# Autodesk Inventor assembly: Assembly8
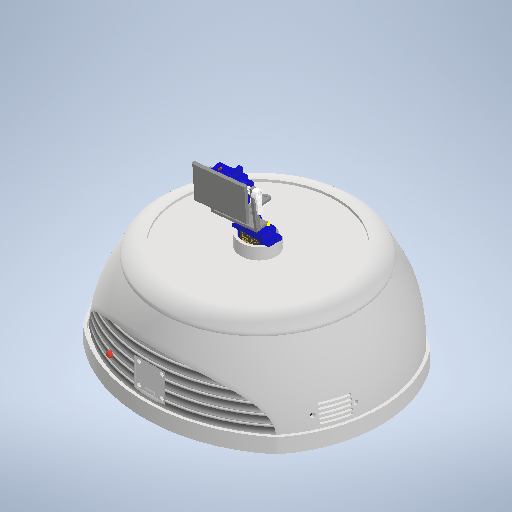
[picture p0: Inventor's stored thumbnail of the model, 512x512]
Saved by Autodesk Inventor 2025.3 (Build 293356030, 356C)
## iProperties
Created: 2026-07-17
Part Number: Assembly8
Document SubType Name: Assembly
Designer: Samuel Correa Vega
Author: Samuel Correa Vega
## Documents named in this file (12)
- C:\Users\Samuel Correa Vega\Documents\Mini-Nathan\Full Robot.iam
- C:\Users\Samuel Correa Vega\Documents\Mini-Nathan\Upper Base.ipt
- C:\Users\Samuel Correa Vega\Documents\ROBOT\Beeper buzzer 3-24V 23dia 11h leaded\Beeper buzzer 3-24V 23dia 11h leaded\Beeper buzzer 3-24V 23dia 11h leaded.ipt
- C:\Users\Samuel Correa Vega\Documents\ROBOT\SG90 - Micro Servo 9g - Tower Pro.1\SG90 - Micro Servo 9g - Tower Pro.1\SG90 - Micro Servo 9g - Tower Pro.1.ipt
- C:\Users\Samuel Correa Vega\Documents\ROBOT\SG90 - Micro Servo 9g - Tower Pro.3\SG90 - Micro Servo 9g - Tower Pro.3\SG90 - Micro Servo 9g - Tower Pro.3.ipt
- C:\Users\Samuel Correa Vega\Documents\Mini-Nathan\Servo's neck.ipt
- C:\Users\Samuel Correa Vega\Documents\ROBOT\SG90 - Micro Servo 9g - Tower Pro.2\SG90 - Micro Servo 9g - Tower Pro.2\SG90 - Micro Servo 9g - Tower Pro.2.ipt
- C:\Users\Samuel Correa Vega\Documents\Mini-Nathan\Sensor Piece.ipt
- C:\Users\Samuel Correa Vega\Documents\Mini-Nathan\Inferior Base.ipt
- C:\Users\Samuel Correa Vega\Documents\ROBOT\red led\red led\red led.ipt
- C:\Users\Samuel Correa Vega\Documents\ROBOT\arduino uno\arduino uno\arduino uno.ipt
- C:\Users\Samuel Correa Vega\Documents\ROBOT\porta pilas AA\porta pilas AA\porta pilas AA.ipt
## Components (12 placed, 11 different names)
1. Upper Base:1 — Mate:1, Flush:1, Mate:2, Mate:3, Mate:17, Angle:3, Mate:20, Mate:21, Mate:22, Mate:23, Angle:5
2. Beeper buzzer 3-24V 23dia 11h leaded:1
3. SG90 - Micro Servo 9g - Tower Pro.1:1 — Mate:3, Mate:4, Mate:5, Mate:6
4. SG90 - Micro Servo 9g - Tower Pro.3:1 — Mate:4, Mate:5, Mate:7, Angle:1
5. Servo's neck:1 — Mate:6, Mate:7, Angle:1, Mate:8, Mate:10, Mate:11, Angle:2
6. SG90 - Micro Servo 9g - Tower Pro.1:2 — Mate:8, Mate:9, Mate:11, Mate:12, Mate:13, Mate:14
7. SG90 - Micro Servo 9g - Tower Pro.2:1 — Mate:9, Mate:10, Angle:2
8. Sensor Piece:1 — Mate:12, Mate:13, Mate:14
9. red led:1 — Mate:20, Mate:21
10. Inferior Base:1 — Mate:22, Mate:27, Mate:28, Angle:6, Symmetry:1, Mate:34, Mate:35
11. arduino uno:1 — Mate:34
12. porta pilas AA:1 — Mate:35
## Relationships (36: Mate 27, Angle 7, Flush 1, Symmetry 1)
- Mate:1: Upper Base:1
- Flush:1: Upper Base:1
- Mate:2: Upper Base:1
- Mate:3: Upper Base:1 ↔ SG90 - Micro Servo 9g - Tower Pro.1:1
- Mate:4: SG90 - Micro Servo 9g - Tower Pro.1:1 ↔ SG90 - Micro Servo 9g - Tower Pro.3:1
- Mate:5: SG90 - Micro Servo 9g - Tower Pro.1:1 ↔ SG90 - Micro Servo 9g - Tower Pro.3:1
- Mate:6: SG90 - Micro Servo 9g - Tower Pro.1:1 ↔ Servo's neck:1
- Mate:7: SG90 - Micro Servo 9g - Tower Pro.3:1 ↔ Servo's neck:1
- Angle:1 (0 deg): SG90 - Micro Servo 9g - Tower Pro.3:1 ↔ Servo's neck:1
- Mate:8: Servo's neck:1 ↔ SG90 - Micro Servo 9g - Tower Pro.1:2
- Mate:9: SG90 - Micro Servo 9g - Tower Pro.1:2 ↔ SG90 - Micro Servo 9g - Tower Pro.2:1
- Mate:10: Servo's neck:1 ↔ SG90 - Micro Servo 9g - Tower Pro.2:1
- Mate:11: Servo's neck:1 ↔ SG90 - Micro Servo 9g - Tower Pro.1:2
- Angle:2 (0 deg): Servo's neck:1 ↔ SG90 - Micro Servo 9g - Tower Pro.2:1
- Mate:12: SG90 - Micro Servo 9g - Tower Pro.1:2 ↔ Sensor Piece:1
- Mate:13: SG90 - Micro Servo 9g - Tower Pro.1:2 ↔ Sensor Piece:1
- Mate:14: SG90 - Micro Servo 9g - Tower Pro.1:2 ↔ Sensor Piece:1
- Mate:17: Upper Base:1
- Angle:3 (0 deg): Upper Base:1
- Angle:4 (90 deg)
- Mate:20: Upper Base:1 ↔ red led:1
- Mate:21: Upper Base:1 ↔ red led:1
- Mate:22: Upper Base:1 ↔ Inferior Base:1
- Mate:23: Upper Base:1
- Angle:5 (0 deg): Upper Base:1
- Mate:26
- Mate:27: Inferior Base:1
- Mate:28: Inferior Base:1
- Mate:31
- Angle:6 (0 deg): Inferior Base:1
- Mate:32
- Angle:7 (0 deg)
- Symmetry:1: Inferior Base:1
- Mate:33
- Mate:34: Inferior Base:1 ↔ arduino uno:1
- Mate:35: Inferior Base:1 ↔ porta pilas AA:1
